# Autodesk Inventor assembly: screw_dfsr03205c1ngc0-2230-p0_ss
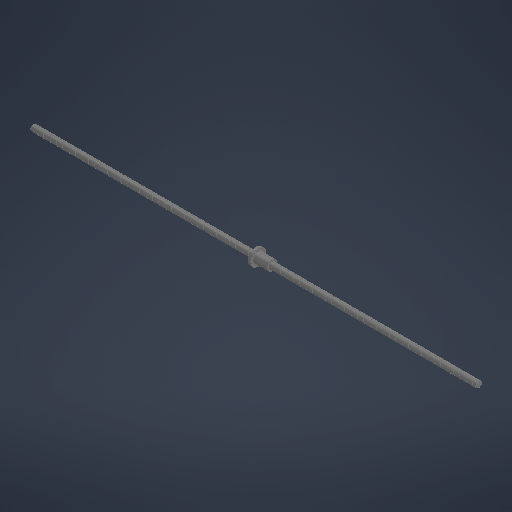
[picture p0: Inventor's stored thumbnail of the model, 512x512]
Saved by Autodesk Inventor 2025 (Build 290162000, 162)
## iProperties
Company: TraceParts S.A.
Created: 2024-05-24
Part Number: screw_dfsr03205c1ngc0-2230-p0_ss
Checked By: TraceParts S.A.
Catalog Web Link: www.traceparts.com
Document SubType Name: Assembly
Designer: TraceParts
Sending System: TraceParts v2
Major Version: 6.0
Minor Version: 0.0
Format Version: 0.0
Product Id: TraceParts v2
REFERENCE: DFSR03205C1NGC0-2230-P0+SS
SUPPLIER: TBI MOTION TECHNOLOGY CO., LTD.
DESIGN: Ball Screw DFSR03205C1NGC0-2230-P0+SS
TraceParts.PartNumber: 33-05092019-058428
TraceParts.PartTitle: Ball Screw / DFS Series
TraceParts.InstanceId: 33-05092019-0584284Y2DHGSJ7ZW40SSRT6QMKUQ7W
TRACEPARTS: TRACEPARTS
TraceParts.PartLanguage: en
TraceParts.PartVersion: 1.0.2
Author: TraceParts
## Documents named in this file (3)
- D:\UNAL\2024-1S\APM\Digital Factory\Linear Guides & Ball Screws\screw_dfsr03205c1ngc0-2230-p0_ss.iam
- D:\UNAL\2024-1S\APM\Digital Factory\Linear Guides & Ball Screws\screw_dfsr03205c1ngc0-2230-p0_ss_01.ipt
- D:\UNAL\2024-1S\APM\Digital Factory\Linear Guides & Ball Screws\screw_dfsr03205c1ngc0-2230-p0_ss_02.ipt
## Components (2 placed, 2 different names)
1. screw_dfsr03205c1ngc0-2230-p0_ss_Temp_1:1 — Cylindrical:1
2. screw_dfsr03205c1ngc0-2230-p0_ss_Temp_2:1 — Cylindrical:1
## Relationships (1: CylindricalJoint 1)
- Cylindrical:1: screw_dfsr03205c1ngc0-2230-p0_ss_Temp_1:1 ↔ screw_dfsr03205c1ngc0-2230-p0_ss_Temp_2:1
